# Autodesk Inventor assembly: Assembly6
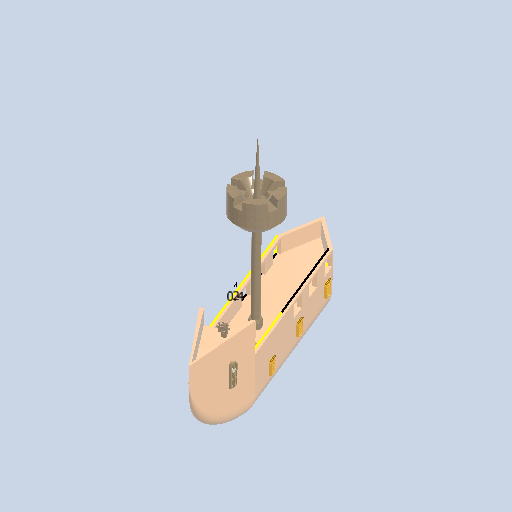
[picture p0: Inventor's stored thumbnail of the model, 512x512]
Saved by Autodesk Inventor 2024.1 (Build 281209000, 209)
## iProperties
Created: 2023-11-09
Part Number: Assembly6
Document SubType Name: Assembly
Designer: luvag
Author: luvag
## Documents named in this file (5)
- C:\Users\luvag\Desktop\Assembly6.iam
- C:\Users\luvag\Desktop\Maitri_door.ipt
- C:\Users\luvag\Desktop\Maitri_Ladder.ipt
- C:\Users\luvag\Desktop\WindowofShip11.ipt
- C:\Users\luvag\Desktop\Assembly4.iam
## Components (9 placed, 4 different names)
1. Maitri_door:1
2. Maitri_Ladder:1
3. WindowofShip:1
4. WindowofShip:2
5. WindowofShip:3
6. WindowofShip:4
7. WindowofShip:5
8. WindowofShip:6
9. Assembly4:1 [sub-assembly]
## Relationships (9: Mate 9)
- [Mate]: Maitri_door:1 ↔ Assembly4:1
- [Mate]: Maitri_Ladder:1 ↔ Assembly4:1
- [Mate]: Maitri_Ladder:1 ↔ Assembly4:1
- [Mate]: WindowofShip:3 ↔ Assembly4:1
- [Mate]: WindowofShip:2 ↔ Assembly4:1
- [Mate]: WindowofShip:1 ↔ Assembly4:1
- [Mate]: WindowofShip:4 ↔ Assembly4:1
- [Mate]: WindowofShip:5 ↔ Assembly4:1
- [Mate]: WindowofShip:6 ↔ Assembly4:1
